# Autodesk Inventor assembly: Potenciometro de Panel
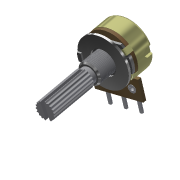
[picture p0: Inventor's stored thumbnail of the model, 180x180]
Saved by Autodesk Inventor 2020 (Build 240168000, 168)
## iProperties
Created: 2016-08-22
Part Number: Potenciometro de Panel
Document SubType Name: Assembly
Designer: Tom
Author: Tom
## Documents named in this file (7)
- C:\Users\Usuario\Desktop\Ensamble Ajust Fino Total + Elect. - Act. 20_10_2020\Componentes Electrónicos\Potenciometro de Panel.iam
- C:\Users\Usuario\Desktop\Ensamble Ajust Fino Total + Elect. - Act. 20_10_2020\Componentes Electrónicos\Potenciometro - Cuerpo.ipt
- C:\Users\Usuario\Desktop\Ensamble Ajust Fino Total + Elect. - Act. 20_10_2020\Componentes Electrónicos\Potenciometro - Cuerpo 2.ipt
- C:\Users\Usuario\Desktop\Ensamble Ajust Fino Total + Elect. - Act. 20_10_2020\Componentes Electrónicos\Potenciometro - Base.ipt
- C:\Users\Usuario\Desktop\Ensamble Ajust Fino Total + Elect. - Act. 20_10_2020\Componentes Electrónicos\Potenciometro - Pata.ipt
- C:\Users\Usuario\Desktop\Ensamble Ajust Fino Total + Elect. - Act. 20_10_2020\Componentes Electrónicos\Potenciometro - Eje.ipt
- C:\Users\Usuario\Desktop\Ensamble Ajust Fino Total + Elect. - Act. 20_10_2020\Componentes Electrónicos\Potenciometro - Arandela.ipt
## Components (8 placed, 6 different names)
1. Part1_panel pot:1 — Mate:3, Mate:4, Angle:3
2. Part3_panel pot:1 — Mate:3, Mate:4, Rigid:1, Mate:6, Angle:2, Angle:3, Rigid:2, Rigid:3, Rotational:2
3. Part4_panel pot:1 — Rigid:1
4. Part4_panel pot:2 — Rigid:2
5. Part4_panel pot:3 — Rigid:3
6. Part2_panel pot:1 — Mate:6, Angle:1, Angle:2, Rotational:2, Rotational:3, Insert:1
7. Part5_panel pot:1 — Rotational:3
8. Part7_panel pot:1 — Insert:1
## Relationships (12: Mate 3, WeldJoint 3, Angle 3, RevoluteJoint 2, Insert 1)
- Mate:3: Part1_panel pot:1 ↔ Part3_panel pot:1
- Mate:4: Part1_panel pot:1 ↔ Part3_panel pot:1
- Rigid:1 [WeldJoint]: Part3_panel pot:1 ↔ Part4_panel pot:1
- Mate:6: Part3_panel pot:1 ↔ Part2_panel pot:1
- Angle:1 (180 deg): Part2_panel pot:1
- Angle:2 (0 deg): Part3_panel pot:1 ↔ Part2_panel pot:1
- Angle:3 (0 deg): Part1_panel pot:1 ↔ Part3_panel pot:1
- Rigid:2 [WeldJoint]: Part3_panel pot:1 ↔ Part4_panel pot:2
- Rigid:3 [WeldJoint]: Part3_panel pot:1 ↔ Part4_panel pot:3
- Rotational:2 [RevoluteJoint]: Part3_panel pot:1 ↔ Part2_panel pot:1
- Rotational:3 [RevoluteJoint]: Part2_panel pot:1 ↔ Part5_panel pot:1
- Insert:1: Part2_panel pot:1 ↔ Part7_panel pot:1
